# Autodesk Inventor assembly: arm
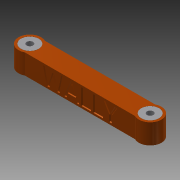
[picture p0: Inventor's stored thumbnail of the model, 180x180]
Saved by Autodesk Inventor 2013 (Build 170138000, 138)
## iProperties
Created: 2013-10-14
Part Number: arm
Document SubType Name: Assembly
Designer: employee
Author: employee
## Documents named in this file (3)
- C:\Users\employee\Desktop\new wally\arm.iam
- C:\Users\employee\Desktop\new wally\xy wall arm.ipt
- C:\Users\employee\Desktop\new wally\608.ipt
## Components (5 placed, 2 different names)
1. xy wall arm:1 — Insert:1, Insert:2, Insert:3, Insert:4
2. 608:1 — Insert:1
3. 608:2 — Insert:4
4. 608:3 — Insert:3
5. 608:4 — Insert:2
## Relationships (4: Insert 4)
- Insert:1: xy wall arm:1 ↔ 608:1
- Insert:2: xy wall arm:1 ↔ 608:4
- Insert:3: xy wall arm:1 ↔ 608:3
- Insert:4: xy wall arm:1 ↔ 608:2
